# Autodesk Inventor assembly: 脚クランク原動節v2
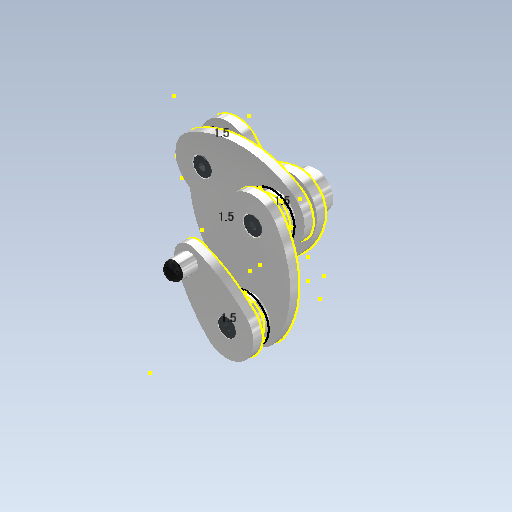
[picture p0: Inventor's stored thumbnail of the model, 512x512]
Saved by Autodesk Inventor 2020.4 (Build 244396000, 396)
## iProperties
Created: 2021-02-21
Part Number: 脚クランク原動節v2
Document SubType Name: Assembly
Designer: AA19065
Mass: 32.3437 g
Surface Area: 166.98 cm^2
Volume: 10.8444 cm^3
Density: 2.98252 g/cm^3
Author: AA19065
## Documents named in this file (10)
- C:\Users\happy\OneDrive\ドキュメント\賢一ファイル\SRDC\試作10-2\アセンブリ\脚クランク原動節v2.iam
- C:\Users\happy\OneDrive\ドキュメント\賢一ファイル\SRDC\試作10-2\脚クランク\原動節v2\原動節0v2.ipt
- C:\Users\happy\OneDrive\ドキュメント\賢一ファイル\SRDC\試作10-2\脚クランク\原動節v2\原動節1-3v2.ipt
- C:\Users\happy\OneDrive\ドキュメント\賢一ファイル\SRDC\試作10-2\脚クランク\原動節v2\原動節4v2.ipt
- C:\Users\happy\OneDrive\ドキュメント\賢一ファイル\SRDC\試作10-2\脚クランク\原動節v2\原動節接続部v2外.ipt
- C:\Users\happy\OneDrive\ドキュメント\賢一ファイル\SRDC\試作10-2\脚クランク\原動節v2\原動節接続部v2内-1.ipt
- C:\Users\happy\OneDrive\ドキュメント\賢一ファイル\SRDC\試作10-2\脚クランク\原動節v2\原動節接続部v2内-2.ipt
- C:\Users\happy\OneDrive\ドキュメント\賢一ファイル\SRDC\試作10-2\ねじ\m3皿ネジ10 (1).ipt
- C:\Users\happy\OneDrive\ドキュメント\賢一ファイル\SRDC\試作10-2\スペーサ\5mm.ipt
- C:\Users\happy\OneDrive\ドキュメント\賢一ファイル\SRDC\試作10-2\ねじ\M3ボタンボルト8.ipt
## Components (25 placed, 9 different names)
1. 原動節0v2:1 — 挿入:13, 挿入:26, 挿入:36, 挿入:37, 挿入:58, 挿入:59, 挿入:60
2. 原動節1-3v2:1 — 挿入:19, 挿入:25, 挿入:30, 挿入:31, 挿入:38, 挿入:39, 挿入:53
3. 原動節4v2:1 — 挿入:34, 挿入:35, 挿入:55, 挿入:56
4. 原動節接続部v2外:1 — 挿入:36, 挿入:37
5. 原動節接続部v2内-1:1 — 挿入:19, 挿入:25, 挿入:48, 挿入:49
6. 原動節接続部v2内-2:1 — 挿入:34, 挿入:35, 挿入:50, 挿入:51
7. 原動節1-3v2:2 — 挿入:17, 挿入:27, 挿入:28, 挿入:29, 挿入:42, 挿入:43, 挿入:54
8. 原動節1-3v2:3 — 挿入:22, 挿入:24, 挿入:32, 挿入:33, 挿入:40, 挿入:41, 挿入:52
9. 原動節接続部v2外:2 — 挿入:38, 挿入:39
10. 原動節接続部v2内-1:2 — 挿入:17, 挿入:27, 挿入:47, 挿入:46
11. 原動節接続部v2内-2:2 — 挿入:28, 挿入:29, 挿入:44, 挿入:45
12. 原動節接続部v2外:3 — 挿入:40, 挿入:41
13. 原動節接続部v2内-1:3 — 挿入:13, 挿入:26, 挿入:44, 挿入:45
14. 原動節接続部v2内-2:3 — 挿入:30, 挿入:31, 挿入:47, 挿入:46
15. 原動節接続部v2外:4 — 挿入:42, 挿入:43
16. 原動節接続部v2内-1:4 — 挿入:22, 挿入:24, 挿入:50, 挿入:51
17. 原動節接続部v2内-2:4 — 挿入:32, 挿入:33, 挿入:48, 挿入:49
18. m3皿ネジ10 (1):1 — 挿入:55
19. m3皿ネジ10 (1):2 — 挿入:54
20. m3皿ネジ10 (1):3 — 挿入:53
21. m3皿ネジ10 (1):4 — 挿入:52
22. 5mm:1 — 挿入:56, 挿入:57
23. M3ボタンボルト8:1 — 挿入:57
24. 原動節接続部v2内-2:5 — 挿入:58, 挿入:59, メイト:1
25. 原動節接続部v2外:5 — 挿入:60, メイト:1
## Relationships (42: Insert 41, Mate 1)
- 挿入:13 [Insert]: 原動節0v2:1 ↔ 原動節接続部v2内-1:3
- 挿入:17 [Insert]: 原動節1-3v2:2 ↔ 原動節接続部v2内-1:2
- 挿入:19 [Insert]: 原動節1-3v2:1 ↔ 原動節接続部v2内-1:1
- 挿入:22 [Insert]: 原動節1-3v2:3 ↔ 原動節接続部v2内-1:4
- 挿入:24 [Insert]: 原動節1-3v2:3 ↔ 原動節接続部v2内-1:4
- 挿入:25 [Insert]: 原動節1-3v2:1 ↔ 原動節接続部v2内-1:1
- 挿入:26 [Insert]: 原動節0v2:1 ↔ 原動節接続部v2内-1:3
- 挿入:27 [Insert]: 原動節1-3v2:2 ↔ 原動節接続部v2内-1:2
- 挿入:28 [Insert]: 原動節1-3v2:2 ↔ 原動節接続部v2内-2:2
- 挿入:29 [Insert]: 原動節1-3v2:2 ↔ 原動節接続部v2内-2:2
- 挿入:30 [Insert]: 原動節1-3v2:1 ↔ 原動節接続部v2内-2:3
- 挿入:31 [Insert]: 原動節1-3v2:1 ↔ 原動節接続部v2内-2:3
- 挿入:32 [Insert]: 原動節1-3v2:3 ↔ 原動節接続部v2内-2:4
- 挿入:33 [Insert]: 原動節1-3v2:3 ↔ 原動節接続部v2内-2:4
- 挿入:34 [Insert]: 原動節4v2:1 ↔ 原動節接続部v2内-2:1
- 挿入:35 [Insert]: 原動節4v2:1 ↔ 原動節接続部v2内-2:1
- 挿入:36 [Insert]: 原動節0v2:1 ↔ 原動節接続部v2外:1
- 挿入:37 [Insert]: 原動節0v2:1 ↔ 原動節接続部v2外:1
- 挿入:38 [Insert]: 原動節1-3v2:1 ↔ 原動節接続部v2外:2
- 挿入:39 [Insert]: 原動節1-3v2:1 ↔ 原動節接続部v2外:2
- 挿入:40 [Insert]: 原動節1-3v2:3 ↔ 原動節接続部v2外:3
- 挿入:41 [Insert]: 原動節1-3v2:3 ↔ 原動節接続部v2外:3
- 挿入:42 [Insert]: 原動節1-3v2:2 ↔ 原動節接続部v2外:4
- 挿入:43 [Insert]: 原動節1-3v2:2 ↔ 原動節接続部v2外:4
- 挿入:44 [Insert] (0.5 mm): 原動節接続部v2内-2:2 ↔ 原動節接続部v2内-1:3
- 挿入:45 [Insert] (0.5 mm): 原動節接続部v2内-2:2 ↔ 原動節接続部v2内-1:3
- 挿入:47 [Insert] (0.5 mm): 原動節接続部v2内-1:2 ↔ 原動節接続部v2内-2:3
- 挿入:46 [Insert] (0.5 mm): 原動節接続部v2内-1:2 ↔ 原動節接続部v2内-2:3
- 挿入:48 [Insert] (0.5 mm): 原動節接続部v2内-1:1 ↔ 原動節接続部v2内-2:4
- 挿入:49 [Insert] (0.5 mm): 原動節接続部v2内-1:1 ↔ 原動節接続部v2内-2:4
- 挿入:50 [Insert] (0.5 mm): 原動節接続部v2内-2:1 ↔ 原動節接続部v2内-1:4
- 挿入:51 [Insert] (0.5 mm): 原動節接続部v2内-2:1 ↔ 原動節接続部v2内-1:4
- 挿入:52 [Insert]: 原動節1-3v2:3 ↔ m3皿ネジ10 (1):4
- 挿入:53 [Insert]: 原動節1-3v2:1 ↔ m3皿ネジ10 (1):3
- 挿入:54 [Insert]: 原動節1-3v2:2 ↔ m3皿ネジ10 (1):2
- 挿入:55 [Insert]: 原動節4v2:1 ↔ m3皿ネジ10 (1):1
- 挿入:56 [Insert]: 原動節4v2:1 ↔ 5mm:1
- 挿入:57 [Insert]: 5mm:1 ↔ M3ボタンボルト8:1
- 挿入:58 [Insert]: 原動節0v2:1 ↔ 原動節接続部v2内-2:5
- 挿入:59 [Insert]: 原動節0v2:1 ↔ 原動節接続部v2内-2:5
- 挿入:60 [Insert]: 原動節0v2:1 ↔ 原動節接続部v2外:5
- メイト:1 [Mate]: 原動節接続部v2内-2:5 ↔ 原動節接続部v2外:5
